# Autodesk Inventor assembly: HACKberry_v1
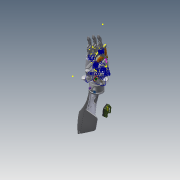
[picture p0: Inventor's stored thumbnail of the model, 180x180]
Saved by Autodesk Inventor 2015 SP1 (Build 190203100, 203)
## iProperties
Created: 2015-02-09
Part Number: HACKberry_v1
Document SubType Name: Assembly
Designer: Yamaura
Author: Yamaura
## Documents named in this file (35)
- C:\Users\Yamaura\Documents\GitHub\HACKberry\HACKberry-hardware\3D\Inventor\HACKberry_v1.iam
- C:\Users\Yamaura\Documents\GitHub\HACKberry\HACKberry-hardware\3D\Inventor\Parts\HB_armMountU03.iam
- C:\Users\Yamaura\Documents\GitHub\HACKberry\HACKberry-hardware\3D\Inventor\Parts\ASV-15MG.ipt
- C:\Users\Yamaura\Documents\GitHub\HACKberry\HACKberry-hardware\3D\Inventor\Parts\HbIndexFinger01.iam
- C:\Users\Yamaura\Documents\GitHub\HACKberry\HACKberry-hardware\3D\Inventor\Parts\HbFinger01.iam
- C:\Users\Yamaura\Documents\GitHub\HACKberry\HACKberry-hardware\3D\Inventor\Parts\HbIndexMotorU01.iam
- C:\Users\Yamaura\Documents\GitHub\HACKberry\HACKberry-hardware\3D\Inventor\Parts\Arduino Micro ASSY.iam
- C:\Users\Yamaura\Documents\GitHub\HACKberry\HACKberry-hardware\3D\Inventor\Parts\ASV-15MGSingleHorn01.ipt
- C:\Users\Yamaura\Documents\GitHub\HACKberry\HACKberry-hardware\3D\Inventor\Parts\HbArduinoMicroShield01.iam
- C:\Users\Yamaura\Documents\GitHub\HACKberry\HACKberry-hardware\3D\Inventor\Parts\HbIndexFinger_flex01.iam
- C:\Users\Yamaura\Documents\GitHub\HACKberry\HACKberry-hardware\3D\Inventor\Parts\HbthumbU01.iam
- C:\Users\Yamaura\Documents\GitHub\HACKberry\HACKberry-hardware\3D\Inventor\Parts\HbFinger_flex02.iam
- C:\Users\Yamaura\Documents\GitHub\HACKberry\HACKberry-hardware\3D\Inventor\Parts\DC-DCconverter.ipt
- C:\Users\Yamaura\Documents\GitHub\HACKberry\HACKberry-hardware\3D\Inventor\Parts\USBmicroConnector01.ipt
- C:\Users\Yamaura\Documents\GitHub\HACKberry\HACKberry-hardware\3D\Inventor\Parts\WasherM2Ph4.3T0.3.ipt
- C:\Users\Yamaura\Documents\GitHub\HACKberry\HACKberry-hardware\3D\Inventor\Parts\ScrewM2L8.ipt
- C:\Users\Yamaura\Documents\GitHub\HACKberry\HACKberry-hardware\3D\Inventor\Parts\MetalCollarPh3L5.ipt
- C:\Users\Yamaura\Documents\GitHub\HACKberry\HACKberry-hardware\3D\Inventor\Parts\ScrewM2L12.ipt
- C:\Users\Yamaura\Documents\GitHub\HACKberry\HACKberry-hardware\3D\Inventor\Parts\HbFingerMainCouplerLink01.ipt
- C:\Users\Yamaura\Documents\GitHub\HACKberry\HACKberry-hardware\3D\Inventor\Parts\HbMiddle-RingCouplerLink01.ipt
- C:\Users\Yamaura\Documents\GitHub\HACKberry\HACKberry-hardware\3D\Inventor\Parts\HbRing-LittleCouplerLink01.ipt
- C:\Users\Yamaura\Documents\GitHub\HACKberry\HACKberry-hardware\3D\Inventor\Parts\UsmBearing01.ipt
- C:\Users\Yamaura\Documents\GitHub\HACKberry\HACKberry-hardware\3D\Inventor\Parts\HbPalmBase03.ipt
- C:\Users\Yamaura\Documents\GitHub\HACKberry\HACKberry-hardware\3D\Inventor\Parts\ScrewM2L6.ipt
- C:\Users\Yamaura\Documents\GitHub\HACKberry\HACKberry-hardware\3D\Inventor\Parts\MJ179PH.ipt
- C:\Users\Yamaura\Documents\GitHub\HACKberry\HACKberry-hardware\3D\Inventor\Parts\ScrewM3L8Btite.ipt
- C:\Users\Yamaura\Documents\GitHub\HACKberry\HACKberry-hardware\3D\Inventor\Parts\HbBackCover02.ipt
- C:\Users\Yamaura\Documents\GitHub\HACKberry\HACKberry-hardware\3D\Inventor\Parts\HbShaftStopperA04.ipt
- C:\Users\Yamaura\Documents\GitHub\HACKberry\HACKberry-hardware\3D\Inventor\Parts\HbShaftStopperB04.ipt
- C:\Users\Yamaura\Documents\GitHub\HACKberry\HACKberry-hardware\3D\Inventor\Parts\HbMaxButton05.ipt
- C:\Users\Yamaura\Documents\GitHub\HACKberry\HACKberry-hardware\3D\Inventor\Parts\HbMinButton05.ipt
- C:\Users\Yamaura\Documents\GitHub\HACKberry\HACKberry-hardware\3D\Inventor\Parts\HbThumbButton05.ipt
- C:\Users\Yamaura\Documents\GitHub\HACKberry\HACKberry-hardware\3D\Inventor\Parts\HbPowerLever05.ipt
- C:\Users\Yamaura\Documents\GitHub\HACKberry\HACKberry-hardware\3D\Inventor\Parts\HbFingerLockButton05.ipt
- C:\Users\Yamaura\Documents\GitHub\HACKberry\HACKberry-hardware\3D\Inventor\Parts\HbSensorU01.iam
## Components (77 placed, 34 different names)
1. ASV-15MG:1 — メイト:13, メイト:44, フラッシュ:36, メイト:45, フラッシュ:156, メイト:170, メイト:207, メイト:210, メイト:215, メイト:216
2. HbIndexFinger01:1 [sub-assembly] — メイト:19, フラッシュ:19, フラッシュ:20, フラッシュ:65, フラッシュ:67, フラッシュ:245, メイト:282
3. HbFinger01:1 [sub-assembly] — メイト:123, フラッシュ:149, メイト:148, フラッシュ:150, メイト:153, メイト:154, メイト:284, メイト:288
4. HbFinger01:2 [sub-assembly] — メイト:83, フラッシュ:84, フラッシュ:85, メイト:102, メイト:111, メイト:117, メイト:109, メイト:269, メイト:285
5. HbFinger01:3 [sub-assembly] — フラッシュ:60, メイト:95, メイト:100, メイト:136, メイト:137, メイト:138, メイト:143, フラッシュ:152, メイト:159
6. HB_armMountU03:1 [sub-assembly] — メイト:25, 角度:4, メイト:254
7. HbIndexMotorU01:1 [sub-assembly] — メイト:36, メイト:37, フラッシュ:229, メイト:244, メイト:245, メイト:246, メイト:247, メイト:248, メイト:249, メイト:250, メイト:251
8. Arduino Micro ASSY:1 [sub-assembly] — フラッシュ:61, フラッシュ:62, メイト:78, メイト:79, フラッシュ:82, メイト:220
9. ASV-15MGSingleHorn01:1 — メイト:44, メイト:126, メイト:165, メイト:215, メイト:227
10. ASV-15MGSingleHorn01:2 — メイト:67, 角度:14, メイト:184, メイト:186, メイト:187, メイト:252, メイト:253
11. HbArduinoMicroShield01:1 [sub-assembly] — フラッシュ:61, フラッシュ:62, メイト:220, メイト:222, メイト:228, メイト:237, メイト:265, メイト:266
12. HbPalmBase03:1 — メイト:222, メイト:228, メイト:252, メイト:254, メイト:235, フラッシュ:234, フラッシュ:235, フラッシュ:241, フラッシュ:242, メイト:261, メイト:262, メイト:275, メイト:277, メイト:278, メイト:279, メイト:280, メイト:281, メイト:83, メイト:282, メイト:290, メイト:291
13. HbIndexFinger_flex01:1 [sub-assembly] — フラッシュ:65, メイト:63, フラッシュ:66, メイト:71, フラッシュ:80
14. HbIndexFinger01:2 [sub-assembly] — フラッシュ:67, メイト:64, 角度:11
15. HbthumbU01:1 [sub-assembly] — 角度:292, メイト:292, メイト:293, メイト:294, フラッシュ:246, 角度:293
16. HbthumbU01:2 [sub-assembly] — メイト:294, フラッシュ:246, 角度:293
17. HbFinger_flex02:1 [sub-assembly] — フラッシュ:71, フラッシュ:191, メイト:191, メイト:193, メイト:194, メイト:197
18. HbFinger_flex02:2 [sub-assembly] — メイト:192, フラッシュ:192, フラッシュ:193, メイト:196
19. HbFinger_flex02:3 [sub-assembly] — フラッシュ:159, フラッシュ:160, メイト:190, メイト:195, メイト:229, メイト:231
20. HbIndexFinger_flex01:2 [sub-assembly] — メイト:71, フラッシュ:80
21. DC-DCconverter:1 — メイト:261, メイト:262
22. USBmicroConnector01:1 — メイト:78, メイト:79, フラッシュ:83
23. WasherM2Ph4.3T0.3:1 — メイト:94, メイト:95, メイト:96
24. WasherM2Ph4.3T0.3:2 — メイト:97, メイト:98, メイト:99
25. WasherM2Ph4.3T0.3:3 — メイト:102, メイト:103, メイト:135, メイト:157
26. WasherM2Ph4.3T0.3:4 — メイト:104, メイト:108, メイト:134
27. WasherM2Ph4.3T0.3:5 — メイト:111, メイト:112, メイト:114, メイト:286
28. WasherM2Ph4.3T0.3:6 — メイト:113, メイト:115, メイト:116
29. WasherM2Ph4.3T0.3:7 — メイト:119, メイト:154, メイト:155, メイト:287, メイト:288, メイト:289
30. WasherM2Ph4.3T0.3:8 — メイト:120, メイト:121, メイト:124
31. ScrewM2L8:1 — メイト:99, メイト:100, メイト:93
32. ScrewM2L8:2 — メイト:108, メイト:109, メイト:105, メイト:134, メイト:135
33. ScrewM2L8:3 — メイト:116, メイト:117, メイト:110, メイト:269, メイト:285
34. ScrewM2L8:4 — メイト:121, メイト:125, メイト:153, メイト:155, メイト:284, メイト:287
35. ScrewM2L8:5 — メイト:129, メイト:131, メイト:132, メイト:130
36. MetalCollarPh3L5:1 — メイト:110, メイト:112, メイト:113, メイト:114, メイト:115, メイト:268
37. MetalCollarPh3L5:2 — メイト:93, メイト:94, メイト:96, メイト:97, メイト:98, メイト:164
38. MetalCollarPh3L5:3 — メイト:103, メイト:104, メイト:105, メイト:156
39. MetalCollarPh3L5:4 — メイト:119, メイト:120, メイト:123, メイト:124, メイト:125, メイト:270
40. MetalCollarPh3L5:5 — メイト:127, メイト:128, メイト:132, メイト:145, メイト:165
41. WasherM2Ph4.3T0.3:9 — メイト:126, メイト:127, メイト:131
42. WasherM2Ph4.3T0.3:10 — メイト:128, メイト:129, メイト:130
43. ScrewM2L12:1 — メイト:136, メイト:137, メイト:160, メイト:161, メイト:162
44. WasherM2Ph4.3T0.3:11 — メイト:138, メイト:140, メイト:162
45. WasherM2Ph4.3T0.3:12 — メイト:143, メイト:146, メイト:161
46. MetalCollarPh3L5:6 — メイト:140, メイト:144, メイト:160
47. HbFingerMainCouplerLink01:1 — メイト:144, メイト:145, メイト:146, メイト:227
48. HbMiddle-RingCouplerLink01:1 — メイト:268, メイト:270, メイト:286, メイト:289
49. HbRing-LittleCouplerLink01:1 — メイト:156, メイト:157, メイト:164, フラッシュ:194
50. ScrewM2L8:7 — メイト:170, メイト:210
51. UsmBearing01:1 — メイト:290, メイト:291, メイト:292, メイト:293
52. ScrewM2L8:9 — メイト:187, メイト:253
53. ScrewM2L8:10 — メイト:184, メイト:186
54. HbIndexFinger01:3 [sub-assembly] — フラッシュ:190, メイト:189, 角度:15
55. HbRing-LittleCouplerLink01:2 — メイト:193, メイト:194, メイト:195, フラッシュ:194
56. HbMiddle-RingCouplerLink01:2 — メイト:196, メイト:197
57. ASV-15MGSingleHorn01:3 — メイト:207, メイト:216, メイト:230
58. HbFingerMainCouplerLink01:2 — メイト:229, メイト:230, メイト:231
59. ScrewM2L6:2 — メイト:235
60. MJ179PH:1 — メイト:237, メイト:242, メイト:243
61. ScrewM3L8Btite:1 — メイト:244, メイト:251
62. ScrewM3L8Btite:2 — メイト:245, メイト:250
63. ScrewM3L8Btite:3 — メイト:246, メイト:248
64. ScrewM3L8Btite:4 — メイト:247, メイト:249
65. HbBackCover02:1 — フラッシュ:230, フラッシュ:241, フラッシュ:242, メイト:273, メイト:274, メイト:276
66. HbShaftStopperA04:1 — フラッシュ:234
67. HbShaftStopperB04:1 — フラッシュ:235
68. HbMaxButton05:1
69. HbMinButton05:1
70. HbThumbButton05:1
71. HbPowerLever05:1
72. HbFingerLockButton05:2 — メイト:265, メイト:266
73. HbSensorU01:1 [sub-assembly]
74. ScrewM2L8:11 — メイト:273, メイト:276, メイト:277
75. ScrewM2L8:12 — メイト:274, メイト:275
76. ScrewM2L8:13 — メイト:278, メイト:280
77. ScrewM2L8:14 — メイト:279, メイト:281
## Relationships (223: Mate 158, Flush 56, Angle 9)
- フラッシュ:1 [Flush] (9.25 mm)
- フラッシュ:2 [Flush] (18.5 mm)
- フラッシュ:3 [Flush] (-18.5 mm)
- フラッシュ:4 [Flush] (-18.5 mm)
- フラッシュ:5 [Flush] (88.4 mm)
- メイト:7 [Mate]
- メイト:8 [Mate]
- フラッシュ:7 [Flush] (-9.25 mm)
- フラッシュ:9 [Flush] (28 mm)
- フラッシュ:10 [Flush] (-7 mm)
- メイト:11 [Mate]
- メイト:12 [Mate]
- メイト:13 [Mate]: ASV-15MG:1
- フラッシュ:16 [Flush] (2.3 mm)
- フラッシュ:17 [Flush] (-10 mm)
- メイト:17 [Mate]
- メイト:18 [Mate]
- フラッシュ:18 [Flush] (9.25 mm)
- メイト:19 [Mate]: HbIndexFinger01:1
- フラッシュ:19 [Flush] (-5 mm): HbIndexFinger01:1
- フラッシュ:20 [Flush]: HbIndexFinger01:1
- メイト:25 [Mate]: HB_armMountU03:1
- 角度:4 [Angle] (0 deg): HB_armMountU03:1
- メイト:26 [Mate]
- 角度:5 [Angle] (-75 deg)
- メイト:30 [Mate]
- 角度:7 [Angle] (90 deg)
- フラッシュ:28 [Flush] (32 mm)
- フラッシュ:30 [Flush] (18.5 mm)
- フラッシュ:31 [Flush] (-24.3 mm)
- フラッシュ:32 [Flush]
- メイト:34 [Mate]
- メイト:35 [Mate]
- メイト:36 [Mate]: HbIndexMotorU01:1
- メイト:37 [Mate]: HbIndexMotorU01:1
- フラッシュ:33 [Flush] (10 mm)
- メイト:38 [Mate]
- メイト:44 [Mate]: ASV-15MG:1 ↔ ASV-15MGSingleHorn01:1
- フラッシュ:35 [Flush] (16.85 mm)
- フラッシュ:36 [Flush]: ASV-15MG:1
- メイト:45 [Mate]: ASV-15MG:1
- フラッシュ:60 [Flush]: HbFinger01:3
- フラッシュ:61 [Flush]: Arduino Micro ASSY:1 ↔ HbArduinoMicroShield01:1
- フラッシュ:62 [Flush]: Arduino Micro ASSY:1 ↔ HbArduinoMicroShield01:1
- フラッシュ:65 [Flush]: HbIndexFinger01:1 ↔ HbIndexFinger_flex01:1
- メイト:63 [Mate]: HbIndexFinger_flex01:1
- フラッシュ:66 [Flush]: HbIndexFinger_flex01:1
- フラッシュ:67 [Flush]: HbIndexFinger01:1 ↔ HbIndexFinger01:2
- メイト:64 [Mate]: HbIndexFinger01:2
- 角度:11 [Angle] (85 deg): HbIndexFinger01:2
- フラッシュ:68 [Flush] (33.5 mm)
- メイト:65 [Mate]
- メイト:66 [Mate]
- メイト:67 [Mate]: ASV-15MGSingleHorn01:2
- フラッシュ:71 [Flush]: HbFinger_flex02:1
- メイト:71 [Mate]: HbIndexFinger_flex01:1 ↔ HbIndexFinger_flex01:2
- フラッシュ:80 [Flush]: HbIndexFinger_flex01:1 ↔ HbIndexFinger_flex01:2
- メイト:78 [Mate]: Arduino Micro ASSY:1 ↔ USBmicroConnector01:1
- メイト:79 [Mate]: Arduino Micro ASSY:1 ↔ USBmicroConnector01:1
- フラッシュ:82 [Flush] (-1.75 mm): Arduino Micro ASSY:1
- フラッシュ:83 [Flush]: USBmicroConnector01:1
- 角度:14 [Angle] (0 deg): ASV-15MGSingleHorn01:2
- メイト:81 [Mate]
- メイト:82 [Mate]
- メイト:83 [Mate]: HbFinger01:2 ↔ HbPalmBase03:1
- フラッシュ:84 [Flush]: HbFinger01:2
- フラッシュ:85 [Flush]: HbFinger01:2
- メイト:93 [Mate]: ScrewM2L8:1 ↔ MetalCollarPh3L5:2
- メイト:94 [Mate]: WasherM2Ph4.3T0.3:1 ↔ MetalCollarPh3L5:2
- メイト:95 [Mate]: HbFinger01:3 ↔ WasherM2Ph4.3T0.3:1
- メイト:96 [Mate]: WasherM2Ph4.3T0.3:1 ↔ MetalCollarPh3L5:2
- メイト:97 [Mate]: WasherM2Ph4.3T0.3:2 ↔ MetalCollarPh3L5:2
- メイト:98 [Mate]: WasherM2Ph4.3T0.3:2 ↔ MetalCollarPh3L5:2
- メイト:99 [Mate]: WasherM2Ph4.3T0.3:2 ↔ ScrewM2L8:1
- メイト:100 [Mate]: HbFinger01:3 ↔ ScrewM2L8:1
- メイト:102 [Mate]: HbFinger01:2 ↔ WasherM2Ph4.3T0.3:3
- メイト:103 [Mate]: WasherM2Ph4.3T0.3:3 ↔ MetalCollarPh3L5:3
- メイト:104 [Mate]: WasherM2Ph4.3T0.3:4 ↔ MetalCollarPh3L5:3
- メイト:105 [Mate]: ScrewM2L8:2 ↔ MetalCollarPh3L5:3
- メイト:108 [Mate]: WasherM2Ph4.3T0.3:4 ↔ ScrewM2L8:2
- メイト:109 [Mate]: HbFinger01:2 ↔ ScrewM2L8:2
- メイト:110 [Mate]: ScrewM2L8:3 ↔ MetalCollarPh3L5:1
- メイト:111 [Mate]: HbFinger01:2 ↔ WasherM2Ph4.3T0.3:5
- メイト:112 [Mate]: WasherM2Ph4.3T0.3:5 ↔ MetalCollarPh3L5:1
- メイト:113 [Mate]: WasherM2Ph4.3T0.3:6 ↔ MetalCollarPh3L5:1
- メイト:114 [Mate]: WasherM2Ph4.3T0.3:5 ↔ MetalCollarPh3L5:1
- メイト:115 [Mate]: WasherM2Ph4.3T0.3:6 ↔ MetalCollarPh3L5:1
- メイト:116 [Mate]: WasherM2Ph4.3T0.3:6 ↔ ScrewM2L8:3
- メイト:117 [Mate]: HbFinger01:2 ↔ ScrewM2L8:3
- メイト:119 [Mate]: WasherM2Ph4.3T0.3:7 ↔ MetalCollarPh3L5:4
- メイト:120 [Mate]: WasherM2Ph4.3T0.3:8 ↔ MetalCollarPh3L5:4
- メイト:121 [Mate]: WasherM2Ph4.3T0.3:8 ↔ ScrewM2L8:4
- メイト:123 [Mate]: HbFinger01:1 ↔ MetalCollarPh3L5:4
- メイト:124 [Mate]: WasherM2Ph4.3T0.3:8 ↔ MetalCollarPh3L5:4
- メイト:125 [Mate]: ScrewM2L8:4 ↔ MetalCollarPh3L5:4
- メイト:126 [Mate]: ASV-15MGSingleHorn01:1 ↔ WasherM2Ph4.3T0.3:9
- メイト:127 [Mate]: MetalCollarPh3L5:5 ↔ WasherM2Ph4.3T0.3:9
- メイト:128 [Mate]: MetalCollarPh3L5:5 ↔ WasherM2Ph4.3T0.3:10
- メイト:129 [Mate]: ScrewM2L8:5 ↔ WasherM2Ph4.3T0.3:10
- メイト:130 [Mate]: ScrewM2L8:5 ↔ WasherM2Ph4.3T0.3:10
- メイト:131 [Mate]: ScrewM2L8:5 ↔ WasherM2Ph4.3T0.3:9
- メイト:132 [Mate]: ScrewM2L8:5 ↔ MetalCollarPh3L5:5
- メイト:134 [Mate]: WasherM2Ph4.3T0.3:4 ↔ ScrewM2L8:2
- メイト:135 [Mate]: WasherM2Ph4.3T0.3:3 ↔ ScrewM2L8:2
- メイト:136 [Mate]: HbFinger01:3 ↔ ScrewM2L12:1
- メイト:137 [Mate]: HbFinger01:3 ↔ ScrewM2L12:1
- メイト:138 [Mate]: HbFinger01:3 ↔ WasherM2Ph4.3T0.3:11
- メイト:140 [Mate]: WasherM2Ph4.3T0.3:11 ↔ MetalCollarPh3L5:6
- メイト:143 [Mate]: HbFinger01:3 ↔ WasherM2Ph4.3T0.3:12
- メイト:144 [Mate]: MetalCollarPh3L5:6 ↔ HbFingerMainCouplerLink01:1
- メイト:145 [Mate]: MetalCollarPh3L5:5 ↔ HbFingerMainCouplerLink01:1
- メイト:146 [Mate] (0.1 mm): WasherM2Ph4.3T0.3:12 ↔ HbFingerMainCouplerLink01:1
- フラッシュ:93 [Flush] (5 mm)
- フラッシュ:149 [Flush]: HbFinger01:1
- メイト:148 [Mate]: HbFinger01:1
- フラッシュ:150 [Flush]: HbFinger01:1
- フラッシュ:151 [Flush] (-5 mm)
- フラッシュ:152 [Flush]: HbFinger01:3
- メイト:153 [Mate]: HbFinger01:1 ↔ ScrewM2L8:4
- メイト:154 [Mate]: HbFinger01:1 ↔ WasherM2Ph4.3T0.3:7
- メイト:155 [Mate]: WasherM2Ph4.3T0.3:7 ↔ ScrewM2L8:4
- メイト:156 [Mate]: MetalCollarPh3L5:3 ↔ HbRing-LittleCouplerLink01:1
- メイト:157 [Mate] (0.1 mm): WasherM2Ph4.3T0.3:3 ↔ HbRing-LittleCouplerLink01:1
- メイト:159 [Mate]: HbFinger01:3
- メイト:160 [Mate]: ScrewM2L12:1 ↔ MetalCollarPh3L5:6
- メイト:161 [Mate]: ScrewM2L12:1 ↔ WasherM2Ph4.3T0.3:12
- メイト:162 [Mate]: ScrewM2L12:1 ↔ WasherM2Ph4.3T0.3:11
- メイト:164 [Mate]: MetalCollarPh3L5:2 ↔ HbRing-LittleCouplerLink01:1
- メイト:165 [Mate]: ASV-15MGSingleHorn01:1 ↔ MetalCollarPh3L5:5
- フラッシュ:156 [Flush] (-11.8 mm): ASV-15MG:1
- メイト:170 [Mate]: ASV-15MG:1 ↔ ScrewM2L8:7
- フラッシュ:159 [Flush]: HbFinger_flex02:3
- フラッシュ:160 [Flush]: HbFinger_flex02:3
- メイト:184 [Mate]: ASV-15MGSingleHorn01:2 ↔ ScrewM2L8:10
- メイト:186 [Mate]: ASV-15MGSingleHorn01:2 ↔ ScrewM2L8:10
- メイト:187 [Mate]: ASV-15MGSingleHorn01:2 ↔ ScrewM2L8:9
- フラッシュ:190 [Flush]: HbIndexFinger01:3
- メイト:189 [Mate]: HbIndexFinger01:3
- 角度:15 [Angle] (0 deg): HbIndexFinger01:3
- メイト:190 [Mate]: HbFinger_flex02:3
- フラッシュ:191 [Flush]: HbFinger_flex02:1
- メイト:191 [Mate]: HbFinger_flex02:1
- メイト:192 [Mate]: HbFinger_flex02:2
- フラッシュ:192 [Flush]: HbFinger_flex02:2
- フラッシュ:193 [Flush]: HbFinger_flex02:2
- メイト:193 [Mate]: HbFinger_flex02:1 ↔ HbRing-LittleCouplerLink01:2
- メイト:194 [Mate]: HbFinger_flex02:1 ↔ HbRing-LittleCouplerLink01:2
- メイト:195 [Mate]: HbFinger_flex02:3 ↔ HbRing-LittleCouplerLink01:2
- フラッシュ:194 [Flush]: HbRing-LittleCouplerLink01:1 ↔ HbRing-LittleCouplerLink01:2
- メイト:196 [Mate]: HbFinger_flex02:2 ↔ HbMiddle-RingCouplerLink01:2
- メイト:197 [Mate]: HbFinger_flex02:1 ↔ HbMiddle-RingCouplerLink01:2
- メイト:203 [Mate]
- 角度:16 [Angle] (90 deg)
- メイト:207 [Mate]: ASV-15MG:1 ↔ ASV-15MGSingleHorn01:3
- メイト:210 [Mate]: ASV-15MG:1 ↔ ScrewM2L8:7
- メイト:215 [Mate]: ASV-15MG:1 ↔ ASV-15MGSingleHorn01:1
- メイト:216 [Mate]: ASV-15MG:1 ↔ ASV-15MGSingleHorn01:3
- メイト:220 [Mate]: Arduino Micro ASSY:1 ↔ HbArduinoMicroShield01:1
- メイト:222 [Mate]: HbArduinoMicroShield01:1 ↔ HbPalmBase03:1
- メイト:227 [Mate]: ASV-15MGSingleHorn01:1 ↔ HbFingerMainCouplerLink01:1
- メイト:228 [Mate]: HbArduinoMicroShield01:1 ↔ HbPalmBase03:1
- メイト:229 [Mate]: HbFinger_flex02:3 ↔ HbFingerMainCouplerLink01:2
- メイト:230 [Mate]: ASV-15MGSingleHorn01:3 ↔ HbFingerMainCouplerLink01:2
- メイト:231 [Mate] (0.15 mm): HbFinger_flex02:3 ↔ HbFingerMainCouplerLink01:2
- メイト:235 [Mate]: HbPalmBase03:1 ↔ ScrewM2L6:2
- メイト:237 [Mate]: HbArduinoMicroShield01:1 ↔ MJ179PH:1
- メイト:242 [Mate] (25.3 mm): MJ179PH:1
- メイト:243 [Mate] (41.4 mm): MJ179PH:1
- フラッシュ:229 [Flush]: HbIndexMotorU01:1
- メイト:244 [Mate]: HbIndexMotorU01:1 ↔ ScrewM3L8Btite:1
- メイト:245 [Mate]: HbIndexMotorU01:1 ↔ ScrewM3L8Btite:2
- メイト:246 [Mate]: HbIndexMotorU01:1 ↔ ScrewM3L8Btite:3
- メイト:247 [Mate]: HbIndexMotorU01:1 ↔ ScrewM3L8Btite:4
- メイト:248 [Mate]: HbIndexMotorU01:1 ↔ ScrewM3L8Btite:3
- メイト:249 [Mate]: HbIndexMotorU01:1 ↔ ScrewM3L8Btite:4
- メイト:250 [Mate]: HbIndexMotorU01:1 ↔ ScrewM3L8Btite:2
- メイト:251 [Mate]: HbIndexMotorU01:1 ↔ ScrewM3L8Btite:1
- メイト:252 [Mate]: ASV-15MGSingleHorn01:2 ↔ HbPalmBase03:1
- メイト:253 [Mate]: ASV-15MGSingleHorn01:2 ↔ ScrewM2L8:9
- フラッシュ:230 [Flush]: HbBackCover02:1
- メイト:254 [Mate]: HB_armMountU03:1 ↔ HbPalmBase03:1
- フラッシュ:234 [Flush]: HbPalmBase03:1 ↔ HbShaftStopperA04:1
- フラッシュ:235 [Flush]: HbPalmBase03:1 ↔ HbShaftStopperB04:1
- フラッシュ:241 [Flush]: HbPalmBase03:1 ↔ HbBackCover02:1
- フラッシュ:242 [Flush]: HbPalmBase03:1 ↔ HbBackCover02:1
- [Mate]: HbArduinoMicroShield01:1 ↔ HbMaxButton05:1
- [Mate]: HbArduinoMicroShield01:1 ↔ HbMinButton05:1
- [Mate]: HbArduinoMicroShield01:1 ↔ HbThumbButton05:1
- [Mate]: HbArduinoMicroShield01:1 ↔ HbMaxButton05:1
- [Flush]: HbMaxButton05:1 ↔ HbMinButton05:1
- [Flush]: HbMinButton05:1 ↔ HbThumbButton05:1
- メイト:261 [Mate]: HbPalmBase03:1 ↔ DC-DCconverter:1
- メイト:262 [Mate]: HbPalmBase03:1 ↔ DC-DCconverter:1
- メイト:265 [Mate]: HbArduinoMicroShield01:1 ↔ HbFingerLockButton05:2
- メイト:266 [Mate]: HbArduinoMicroShield01:1 ↔ HbFingerLockButton05:2
- メイト:268 [Mate]: MetalCollarPh3L5:1 ↔ HbMiddle-RingCouplerLink01:1
- メイト:269 [Mate]: HbFinger01:2 ↔ ScrewM2L8:3
- メイト:270 [Mate]: MetalCollarPh3L5:4 ↔ HbMiddle-RingCouplerLink01:1
- メイト:273 [Mate]: HbBackCover02:1 ↔ ScrewM2L8:11
- メイト:274 [Mate]: HbBackCover02:1 ↔ ScrewM2L8:12
- メイト:275 [Mate]: HbPalmBase03:1 ↔ ScrewM2L8:12
- メイト:276 [Mate]: HbBackCover02:1 ↔ ScrewM2L8:11
- メイト:277 [Mate]: HbPalmBase03:1 ↔ ScrewM2L8:11
- メイト:278 [Mate]: HbPalmBase03:1 ↔ ScrewM2L8:13
- メイト:279 [Mate]: HbPalmBase03:1 ↔ ScrewM2L8:14
- メイト:280 [Mate]: HbPalmBase03:1 ↔ ScrewM2L8:13
- メイト:281 [Mate]: HbPalmBase03:1 ↔ ScrewM2L8:14
- フラッシュ:245 [Flush] (8 mm): HbIndexFinger01:1
- メイト:282 [Mate]: HbIndexFinger01:1 ↔ HbPalmBase03:1
- メイト:284 [Mate]: HbFinger01:1 ↔ ScrewM2L8:4
- メイト:285 [Mate]: HbFinger01:2 ↔ ScrewM2L8:3
- メイト:286 [Mate]: WasherM2Ph4.3T0.3:5 ↔ HbMiddle-RingCouplerLink01:1
- メイト:287 [Mate]: WasherM2Ph4.3T0.3:7 ↔ ScrewM2L8:4
- メイト:288 [Mate]: HbFinger01:1 ↔ WasherM2Ph4.3T0.3:7
- メイト:289 [Mate] (0.1 mm): WasherM2Ph4.3T0.3:7 ↔ HbMiddle-RingCouplerLink01:1
- メイト:290 [Mate]: HbPalmBase03:1 ↔ UsmBearing01:1
- 角度:292 [Angle] (180 deg): HbthumbU01:1
- メイト:291 [Mate]: HbPalmBase03:1 ↔ UsmBearing01:1
- メイト:292 [Mate]: HbthumbU01:1 ↔ UsmBearing01:1
- メイト:293 [Mate]: HbthumbU01:1 ↔ UsmBearing01:1
- メイト:294 [Mate]: HbthumbU01:1 ↔ HbthumbU01:2
- フラッシュ:246 [Flush]: HbthumbU01:1 ↔ HbthumbU01:2
- 角度:293 [Angle] (65 deg): HbthumbU01:1 ↔ HbthumbU01:2
